# Autodesk Inventor assembly: Передача с помощью зубчатых ремней
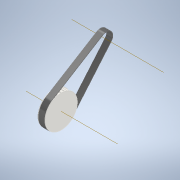
[picture p0: Inventor's stored thumbnail of the model, 180x180]
Saved by Autodesk Inventor 2021 (Build 250183000, 183)
## iProperties
Created: 2021-06-15
Part Number: Передача с помощью зубчатых ремней
Document SubType Name: Assembly
Designer: panda
ClientObjectVersion: 1
Author: panda
## Documents named in this file (3)
- C:\Users\panda\Desktop\vkrb\сборка\Сборка\Мастер проектирования\Передача с помощью зубчатых ремней1.iam
- C:\Users\panda\Desktop\vkrb\сборка\Сборка\Мастер проектирования\Зубчатый ремень1.ipt
- C:\Users\panda\Desktop\vkrb\сборка\Сборка\Мастер проектирования\Синхронный шкив21.ipt
## Components (2 placed, 2 different names)
1. Зубчатый ремень:1 — Заподлицо:1, Совмещение:1, Совмещение:2
2. Синхронный шкив2:1 — Заподлицо:1, Совмещение:1, Совмещение:2
## Relationships (3: Mate 2, Flush 1)
- Заподлицо:1 [Flush]: Зубчатый ремень:1 ↔ Синхронный шкив2:1
- Совмещение:1 [Mate]: Зубчатый ремень:1 ↔ Синхронный шкив2:1
- Совмещение:2 [Mate]: Зубчатый ремень:1 ↔ Синхронный шкив2:1
